# Autodesk Inventor assembly: 조립품3
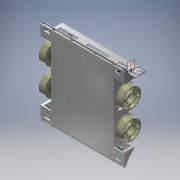
[picture p0: Inventor's stored thumbnail of the model, 180x180]
Saved by Autodesk Inventor 2017 (Build 210142000, 142)
## iProperties
Part Number: 조립품3
Material: 일반
Document SubType Name: Assembly
Designer: minom
Mass: 2146.86 g
Surface Area: 6194.86 cm^2
Volume: 942.713 cm^3
Density: 2.27732 g/cm^3
Author: minom
## Documents named in this file (24)
- C:\Users\minom\Documents\Inventor\Projects\2017 IRC Sumo Mino ver.2\조립품3.iam
- C:\Users\minom\Documents\Inventor\Projects\2017 IRC Sumo Mino ver.2\옆판_오른쪽.ipt
- C:\Users\minom\Documents\Inventor\Projects\2017 IRC Sumo Mino ver.2\옆판_왼쪽.ipt
- C:\Users\minom\Documents\Inventor\Projects\2017 IRC Sumo Mino ver.2\앞뒷판_밑.ipt
- C:\Users\minom\Documents\Inventor\Projects\2017 IRC Sumo Mino ver.2\앞뒷판_중간.ipt
- C:\Users\minom\Documents\Inventor\Projects\2017 IRC Sumo Mino ver.2\IG-42GM_motor.ipt
- C:\Users\minom\Documents\Inventor\Projects\2017 IRC Sumo Mino ver.2\바퀴.ipt
- C:\Users\minom\Documents\Inventor\Projects\2017 IRC Sumo Mino ver.2\바퀴8PI.ipt
- C:\Users\minom\Documents\Inventor\Projects\2017 IRC Sumo Mino ver.2\ATP25XL025-A-N8-KC90-QFC20-M3-FC45_0-TPC3_b.ipt
- C:\Users\minom\Documents\Inventor\Projects\2017 IRC Sumo Mino ver.2\IR모듈.ipt
- C:\Users\minom\Documents\Inventor\Projects\2017 IRC Sumo Mino ver.2\앞판센서막이.ipt
- C:\Users\minom\Documents\Inventor\Projects\2017 IRC Sumo Mino ver.2\밑판_수정.ipt
- C:\Users\minom\Documents\Inventor\Projects\2017 IRC Sumo Mino ver.2\FL6700ZZ.ipt
- C:\Users\minom\Documents\Inventor\Projects\2017 IRC Sumo Mino ver.2\10PI축.ipt
- C:\Users\minom\Documents\Inventor\Projects\2017 IRC Sumo Mino ver.2\베어링받침대.ipt
- C:\Users\minom\Documents\Inventor\Projects\2017 IRC Sumo Mino ver.2\ATP25XL025-A-N10-KC90-QFC20-M3-FC45_0-TPC3_b.ipt
- C:\Users\minom\Documents\Inventor\Projects\2017 IRC Sumo Mino ver.2\모터받침대.ipt
- C:\Users\minom\Documents\Inventor\Projects\2017 IRC Sumo Mino ver.2\CdS모듈.ipt
- C:\Users\minom\Documents\Inventor\Projects\2017 IRC Sumo Mino ver.2\앞판센서막이_오른쪽.ipt
- C:\Users\minom\Documents\Inventor\Projects\2017 IRC Sumo Mino ver.2\8060모터드라이브.ipt
- C:\Users\minom\Documents\Inventor\Projects\2017 IRC Sumo Mino ver.2\앞뒷판_위_수정.ipt
- C:\Users\minom\Documents\Inventor\Projects\2017 IRC Sumo Mino ver.2\대각선PSD받침대.ipt
- C:\Users\minom\Documents\Inventor\Projects\2017 IRC Sumo Mino ver.2\앞뒷면PSD받침대_수정.ipt
- C:\Users\minom\Documents\Inventor\Projects\2017 IRC Sumo Mino ver.2\칼팁중간받침대.ipt
## Components (49 placed, 23 different names)
1. 옆판_오른쪽:1 — 메이트:30, 메이트:31, 메이트:32, 메이트:58, 메이트:59, 메이트:60, 메이트:62, 메이트:63, 메이트:64, 메이트:92, 메이트:93, 메이트:105, 메이트:106, 메이트:121, 메이트:183, 메이트:231, 메이트:259, 메이트:260, 메이트:261, 메이트:262
2. 옆판_왼쪽:1 — 메이트:29, 메이트:45, 메이트:46, 메이트:107, 메이트:108, 메이트:120, 메이트:140, 메이트:148, 메이트:150, 메이트:168, 메이트:185, 메이트:235
3. 앞뒷판_밑:1 — 메이트:168, 메이트:169, 메이트:170, 메이트:223, 메이트:225, 메이트:254, 메이트:257
4. 앞뒷판_밑:2 — 메이트:58, 메이트:62, 메이트:63, 메이트:64, 메이트:66, 메이트:88, 메이트:202, 메이트:218, 메이트:221, 메이트:248, 메이트:251
5. 앞뒷판_중간:1 — 메이트:59, 메이트:60, 메이트:67, 메이트:97, 메이트:262
6. 앞뒷판_중간:2 — 메이트:148, 메이트:149, 메이트:150
7. IG-42GM_motor:1 — 메이트:45, 메이트:46, 메이트:47, 메이트:48, 메이트:245
8. IG-42GM_motor:2 — 메이트:30, 메이트:31, 메이트:33, 메이트:127, 메이트:243
9. 바퀴:1 — 메이트:125
10. 바퀴8PI:1 — 메이트:34, 메이트:127
11. 바퀴:2 — 메이트:124
12. 바퀴8PI:2 — 메이트:48, 메이트:49
13. ATP25XL025-A-N8-KC90-QFC20-M3-FC45_0-TPC3_b:1 — 메이트:29, 메이트:47, 메이트:49
14. ATP25XL025-A-N8-KC90-QFC20-M3-FC45_0-TPC3_b:2 — 메이트:32, 메이트:33, 메이트:34
15. IR모듈:1 — 메이트:102, 플러쉬:8
16. IR모듈:2 — 메이트:80, 메이트:99, 메이트:258, 플러쉬:17
17. IR모듈:3 — 메이트:101, 플러쉬:5
18. IR모듈:4 — 메이트:84, 메이트:103, 플러쉬:7
19. 앞판센서막이:1 — 메이트:66, 메이트:67, 메이트:80, 메이트:88, 메이트:97
20. 앞판센서막이:3 — 메이트:84, 메이트:149, 메이트:151, 메이트:169, 메이트:170
21. 밑판_수정:1 — 메이트:92, 메이트:93, 메이트:99, 메이트:101, 플러쉬:5, 메이트:102, 메이트:103, 플러쉬:7, 플러쉬:8, 메이트:132, 메이트:133, 메이트:134, 메이트:135, 메이트:136, 메이트:137, 메이트:151, 메이트:167, 플러쉬:13, 메이트:184, 플러쉬:14, 메이트:202, 메이트:219, 메이트:220, 메이트:222, 메이트:224, 메이트:236, 메이트:237, 메이트:238, 메이트:239, 메이트:240, 메이트:241, 메이트:242, 메이트:244, 메이트:246, 메이트:247, 메이트:249, 메이트:250, 메이트:252, 메이트:253, 메이트:255, 메이트:256, 메이트:258, 플러쉬:17
22. FL6700ZZ:1 — 메이트:107, 메이트:108, 플러쉬:10, 메이트:109, 메이트:118
23. FL6700ZZ:2 — 플러쉬:10, 메이트:109, 플러쉬:16
24. FL6700ZZ:3 — 메이트:105, 메이트:106, 플러쉬:9, 메이트:110
25. FL6700ZZ:4 — 플러쉬:9, 메이트:110, 플러쉬:15
26. 10PI축:1 — 메이트:229, 플러쉬:15, 메이트:230
27. 10PI축:2 — 메이트:118, 메이트:232, 메이트:234, 플러쉬:16
28. 베어링받침대:1 — 메이트:135, 메이트:136, 메이트:137, 메이트:233
29. 베어링받침대:2 — 메이트:132, 메이트:133, 메이트:134, 메이트:227, 메이트:228
30. ATP25XL025-A-N10-KC90-QFC20-M3-FC45_0-TPC3_b:1 — 메이트:120, 메이트:124
31. ATP25XL025-A-N10-KC90-QFC20-M3-FC45_0-TPC3_b:2 — 메이트:121, 메이트:125
32. 모터받침대:1 — 메이트:140, 메이트:244, 메이트:245
33. 모터받침대:2 — 메이트:242, 메이트:243
34. CdS모듈:1 — 메이트:167, 플러쉬:13, 메이트:183
35. CdS모듈:2 — 메이트:184, 플러쉬:14, 메이트:185
36. 앞판센서막이_오른쪽:1 — 메이트:218, 메이트:219, 메이트:220, 메이트:221
37. 앞판센서막이_오른쪽:2 — 메이트:222, 메이트:223, 메이트:224, 메이트:225
38. 8060모터드라이브:1
39. FL6700ZZ:5 — 메이트:227, 메이트:228, 메이트:229
40. FL6700ZZ:6 — 메이트:230, 메이트:231
41. FL6700ZZ:7 — 메이트:232, 메이트:233
42. FL6700ZZ:8 — 메이트:234, 메이트:235
43. 앞뒷판_위_수정:1 — 메이트:259, 메이트:260, 메이트:261
44. 대각선PSD받침대:1 — 메이트:236, 메이트:237, 메이트:238
45. 앞뒷면PSD받침대_수정:1 — 메이트:239, 메이트:240, 메이트:241
46. 칼팁중간받침대:1 — 메이트:246, 메이트:247, 메이트:248
47. 칼팁중간받침대:2 — 메이트:249, 메이트:250, 메이트:251
48. 칼팁중간받침대:3 — 메이트:252, 메이트:253, 메이트:254
49. 칼팁중간받침대:4 — 메이트:255, 메이트:256, 메이트:257
## Relationships (114: Mate 104, Flush 10)
- 메이트:29 [Mate] (3 mm): 옆판_왼쪽:1 ↔ ATP25XL025-A-N8-KC90-QFC20-M3-FC45_0-TPC3_b:1
- 메이트:30 [Mate]: 옆판_오른쪽:1 ↔ IG-42GM_motor:2
- 메이트:31 [Mate]: 옆판_오른쪽:1 ↔ IG-42GM_motor:2
- 메이트:32 [Mate] (3 mm): 옆판_오른쪽:1 ↔ ATP25XL025-A-N8-KC90-QFC20-M3-FC45_0-TPC3_b:2
- 메이트:33 [Mate]: IG-42GM_motor:2 ↔ ATP25XL025-A-N8-KC90-QFC20-M3-FC45_0-TPC3_b:2
- 메이트:34 [Mate]: 바퀴8PI:1 ↔ ATP25XL025-A-N8-KC90-QFC20-M3-FC45_0-TPC3_b:2
- 메이트:45 [Mate]: 옆판_왼쪽:1 ↔ IG-42GM_motor:1
- 메이트:46 [Mate]: 옆판_왼쪽:1 ↔ IG-42GM_motor:1
- 메이트:47 [Mate]: IG-42GM_motor:1 ↔ ATP25XL025-A-N8-KC90-QFC20-M3-FC45_0-TPC3_b:1
- 메이트:48 [Mate]: IG-42GM_motor:1 ↔ 바퀴8PI:2
- 메이트:49 [Mate]: 바퀴8PI:2 ↔ ATP25XL025-A-N8-KC90-QFC20-M3-FC45_0-TPC3_b:1
- 메이트:58 [Mate] (0.1 mm): 옆판_오른쪽:1 ↔ 앞뒷판_밑:2
- 메이트:59 [Mate] (0.1 mm): 옆판_오른쪽:1 ↔ 앞뒷판_중간:1
- 메이트:60 [Mate]: 옆판_오른쪽:1 ↔ 앞뒷판_중간:1
- 메이트:62 [Mate] (0.1 mm): 옆판_오른쪽:1 ↔ 앞뒷판_밑:2
- 메이트:63 [Mate]: 옆판_오른쪽:1 ↔ 앞뒷판_밑:2
- 메이트:64 [Mate]: 옆판_오른쪽:1 ↔ 앞뒷판_밑:2
- 메이트:66 [Mate] (0.1 mm): 앞뒷판_밑:2 ↔ 앞판센서막이:1
- 메이트:67 [Mate]: 앞뒷판_중간:1 ↔ 앞판센서막이:1
- 메이트:80 [Mate] (8 mm): IR모듈:2 ↔ 앞판센서막이:1
- 메이트:84 [Mate] (8 mm): IR모듈:4 ↔ 앞판센서막이:3
- 메이트:88 [Mate]: 앞뒷판_밑:2 ↔ 앞판센서막이:1
- 메이트:92 [Mate] (0.1 mm): 옆판_오른쪽:1 ↔ 밑판_수정:1
- 메이트:93 [Mate]: 옆판_오른쪽:1 ↔ 밑판_수정:1
- 메이트:97 [Mate] (1 mm): 앞뒷판_중간:1 ↔ 앞판센서막이:1
- 메이트:99 [Mate] (3 mm): IR모듈:2 ↔ 밑판_수정:1
- 메이트:101 [Mate] (6 mm): IR모듈:3 ↔ 밑판_수정:1
- 플러쉬:5 [Flush] (1 mm): IR모듈:3 ↔ 밑판_수정:1
- 메이트:102 [Mate] (6 mm): IR모듈:1 ↔ 밑판_수정:1
- 메이트:103 [Mate] (6 mm): IR모듈:4 ↔ 밑판_수정:1
- 플러쉬:7 [Flush] (1 mm): IR모듈:4 ↔ 밑판_수정:1
- 플러쉬:8 [Flush] (1 mm): IR모듈:1 ↔ 밑판_수정:1
- 메이트:105 [Mate]: 옆판_오른쪽:1 ↔ FL6700ZZ:3
- 메이트:106 [Mate]: 옆판_오른쪽:1 ↔ FL6700ZZ:3
- 메이트:107 [Mate]: 옆판_왼쪽:1 ↔ FL6700ZZ:1
- 메이트:108 [Mate]: 옆판_왼쪽:1 ↔ FL6700ZZ:1
- 플러쉬:9 [Flush] (45 mm): FL6700ZZ:3 ↔ FL6700ZZ:4
- 플러쉬:10 [Flush] (45 mm): FL6700ZZ:1 ↔ FL6700ZZ:2
- 메이트:109 [Mate]: FL6700ZZ:1 ↔ FL6700ZZ:2
- 메이트:110 [Mate]: FL6700ZZ:3 ↔ FL6700ZZ:4
- 메이트:118 [Mate]: FL6700ZZ:1 ↔ 10PI축:2
- 메이트:120 [Mate] (3 mm): 옆판_왼쪽:1 ↔ ATP25XL025-A-N10-KC90-QFC20-M3-FC45_0-TPC3_b:1
- 메이트:121 [Mate] (3 mm): 옆판_오른쪽:1 ↔ ATP25XL025-A-N10-KC90-QFC20-M3-FC45_0-TPC3_b:2
- 메이트:124 [Mate]: 바퀴:2 ↔ ATP25XL025-A-N10-KC90-QFC20-M3-FC45_0-TPC3_b:1
- 메이트:125 [Mate]: 바퀴:1 ↔ ATP25XL025-A-N10-KC90-QFC20-M3-FC45_0-TPC3_b:2
- 메이트:127 [Mate]: IG-42GM_motor:2 ↔ 바퀴8PI:1
- 메이트:132 [Mate]: 밑판_수정:1 ↔ 베어링받침대:2
- 메이트:133 [Mate] (0.1 mm): 밑판_수정:1 ↔ 베어링받침대:2
- 메이트:134 [Mate] (0.1 mm): 밑판_수정:1 ↔ 베어링받침대:2
- 메이트:135 [Mate]: 밑판_수정:1 ↔ 베어링받침대:1
- 메이트:136 [Mate] (0.1 mm): 밑판_수정:1 ↔ 베어링받침대:1
- 메이트:137 [Mate] (0.1 mm): 밑판_수정:1 ↔ 베어링받침대:1
- 메이트:140 [Mate] (80 mm): 옆판_왼쪽:1 ↔ 모터받침대:1
- 메이트:148 [Mate] (0.1 mm): 옆판_왼쪽:1 ↔ 앞뒷판_중간:2
- 메이트:149 [Mate]: 앞뒷판_중간:2 ↔ 앞판센서막이:3
- 메이트:150 [Mate] (1 mm): 옆판_왼쪽:1 ↔ 앞뒷판_중간:2
- 메이트:151 [Mate]: 앞판센서막이:3 ↔ 밑판_수정:1
- 메이트:167 [Mate] (2 mm): 밑판_수정:1 ↔ CdS모듈:1
- 플러쉬:13 [Flush] (1 mm): 밑판_수정:1 ↔ CdS모듈:1
- 메이트:168 [Mate]: 옆판_왼쪽:1 ↔ 앞뒷판_밑:1
- 메이트:169 [Mate] (0.1 mm): 앞뒷판_밑:1 ↔ 앞판센서막이:3
- 메이트:170 [Mate]: 앞뒷판_밑:1 ↔ 앞판센서막이:3
- 메이트:183 [Mate] (95.9 mm): 옆판_오른쪽:1 ↔ CdS모듈:1
- 메이트:184 [Mate] (2 mm): 밑판_수정:1 ↔ CdS모듈:2
- 플러쉬:14 [Flush] (1 mm): 밑판_수정:1 ↔ CdS모듈:2
- 메이트:185 [Mate] (95.9 mm): 옆판_왼쪽:1 ↔ CdS모듈:2
- 메이트:202 [Mate] (10 mm): 앞뒷판_밑:2 ↔ 밑판_수정:1
- 메이트:218 [Mate]: 앞뒷판_밑:2 ↔ 앞판센서막이_오른쪽:1
- 메이트:219 [Mate] (0.1 mm): 밑판_수정:1 ↔ 앞판센서막이_오른쪽:1
- 메이트:220 [Mate]: 밑판_수정:1 ↔ 앞판센서막이_오른쪽:1
- 메이트:221 [Mate]: 앞뒷판_밑:2 ↔ 앞판센서막이_오른쪽:1
- 메이트:222 [Mate] (0.1 mm): 밑판_수정:1 ↔ 앞판센서막이_오른쪽:2
- 메이트:223 [Mate]: 앞뒷판_밑:1 ↔ 앞판센서막이_오른쪽:2
- 메이트:224 [Mate]: 밑판_수정:1 ↔ 앞판센서막이_오른쪽:2
- 메이트:225 [Mate]: 앞뒷판_밑:1 ↔ 앞판센서막이_오른쪽:2
- 메이트:227 [Mate]: 베어링받침대:2 ↔ FL6700ZZ:5
- 메이트:228 [Mate]: 베어링받침대:2 ↔ FL6700ZZ:5
- 메이트:229 [Mate]: 10PI축:1 ↔ FL6700ZZ:5
- 플러쉬:15 [Flush] (-9 mm): FL6700ZZ:4 ↔ 10PI축:1
- 메이트:230 [Mate]: 10PI축:1 ↔ FL6700ZZ:6
- 메이트:231 [Mate]: 옆판_오른쪽:1 ↔ FL6700ZZ:6
- 메이트:232 [Mate]: 10PI축:2 ↔ FL6700ZZ:7
- 메이트:233 [Mate]: 베어링받침대:1 ↔ FL6700ZZ:7
- 메이트:234 [Mate]: 10PI축:2 ↔ FL6700ZZ:8
- 메이트:235 [Mate]: 옆판_왼쪽:1 ↔ FL6700ZZ:8
- 플러쉬:16 [Flush] (-9 mm): FL6700ZZ:2 ↔ 10PI축:2
- 메이트:236 [Mate]: 밑판_수정:1 ↔ 대각선PSD받침대:1
- 메이트:237 [Mate]: 밑판_수정:1 ↔ 대각선PSD받침대:1
- 메이트:238 [Mate]: 밑판_수정:1 ↔ 대각선PSD받침대:1
- 메이트:239 [Mate]: 밑판_수정:1 ↔ 앞뒷면PSD받침대_수정:1
- 메이트:240 [Mate]: 밑판_수정:1 ↔ 앞뒷면PSD받침대_수정:1
- 메이트:241 [Mate]: 밑판_수정:1 ↔ 앞뒷면PSD받침대_수정:1
- 메이트:242 [Mate]: 밑판_수정:1 ↔ 모터받침대:2
- 메이트:243 [Mate]: IG-42GM_motor:2 ↔ 모터받침대:2
- 메이트:244 [Mate]: 밑판_수정:1 ↔ 모터받침대:1
- 메이트:245 [Mate]: IG-42GM_motor:1 ↔ 모터받침대:1
- 메이트:246 [Mate]: 밑판_수정:1 ↔ 칼팁중간받침대:1
- 메이트:247 [Mate] (0.1 mm): 밑판_수정:1 ↔ 칼팁중간받침대:1
- 메이트:248 [Mate]: 앞뒷판_밑:2 ↔ 칼팁중간받침대:1
- 메이트:249 [Mate]: 밑판_수정:1 ↔ 칼팁중간받침대:2
- 메이트:250 [Mate] (0.1 mm): 밑판_수정:1 ↔ 칼팁중간받침대:2
- 메이트:251 [Mate]: 앞뒷판_밑:2 ↔ 칼팁중간받침대:2
- 메이트:252 [Mate]: 밑판_수정:1 ↔ 칼팁중간받침대:3
- 메이트:253 [Mate] (0.1 mm): 밑판_수정:1 ↔ 칼팁중간받침대:3
- 메이트:254 [Mate]: 앞뒷판_밑:1 ↔ 칼팁중간받침대:3
- 메이트:255 [Mate]: 밑판_수정:1 ↔ 칼팁중간받침대:4
- 메이트:256 [Mate] (0.1 mm): 밑판_수정:1 ↔ 칼팁중간받침대:4
- 메이트:257 [Mate]: 앞뒷판_밑:1 ↔ 칼팁중간받침대:4
- 메이트:258 [Mate] (3 mm): IR모듈:2 ↔ 밑판_수정:1
- 플러쉬:17 [Flush] (7 mm): IR모듈:2 ↔ 밑판_수정:1
- 메이트:259 [Mate]: 옆판_오른쪽:1 ↔ 앞뒷판_위_수정:1
- 메이트:260 [Mate] (0.1 mm): 옆판_오른쪽:1 ↔ 앞뒷판_위_수정:1
- 메이트:261 [Mate]: 옆판_오른쪽:1 ↔ 앞뒷판_위_수정:1
- 메이트:262 [Mate] (1 mm): 옆판_오른쪽:1 ↔ 앞뒷판_중간:1
